# Autodesk Inventor assembly: Wine Rack and Light Shelf Assembly
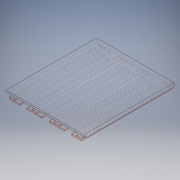
[picture p0: Inventor's stored thumbnail of the model, 180x180]
Saved by Autodesk Inventor 2016 (Build 200138000, 138)
## iProperties
Created: 2017-11-04
Part Number: Wine Rack and Light Shelf Assembly
Document SubType Name: Assembly
Designer: mathaetaes
Author: mathaetaes
## Documents named in this file (4)
- E:\Projects\3D Printer\printer projects\My Designs\Bar Cabinet 2.2.2018\Wine Rack and Light Shelf Assembly Left.iam
- E:\Projects\3D Printer\printer projects\My Designs\Bar Cabinet 2.2.2018\Wine Glass Rack Edge.iam
- E:\Projects\3D Printer\printer projects\My Designs\Bar Cabinet 2.2.2018\Wine Glass Rack Middle.iam
- E:\Projects\3D Printer\printer projects\My Designs\Bar Cabinet 2.2.2018\Horizontal Shelf with Lights Left.ipt
## Components (5 placed, 3 different names)
1. Wine Glass Rack Edge:1 [sub-assembly] — Flush:5, Flush:12, Mate:1
2. Wine Glass Rack Middle:1 [sub-assembly] — Flush:6, Flush:11, Mate:2
3. Wine Glass Rack Edge:2 [sub-assembly] — Flush:8, Flush:9, Mate:4
4. Wine Glass Rack Middle:2 [sub-assembly] — Flush:7, Flush:10, Mate:3
5. Horizontal Shelf with Lights Left:1 — Flush:5, Flush:6, Flush:7, Flush:8, Flush:9, Flush:10, Flush:11, Flush:12, Mate:1, Mate:2, Mate:3, Mate:4
## Relationships (12: Flush 8, Mate 4)
- Flush:5: Wine Glass Rack Edge:1 ↔ Horizontal Shelf with Lights Left:1
- Flush:6: Wine Glass Rack Middle:1 ↔ Horizontal Shelf with Lights Left:1
- Flush:7: Wine Glass Rack Middle:2 ↔ Horizontal Shelf with Lights Left:1
- Flush:8: Wine Glass Rack Edge:2 ↔ Horizontal Shelf with Lights Left:1
- Flush:9: Wine Glass Rack Edge:2 ↔ Horizontal Shelf with Lights Left:1
- Flush:10: Wine Glass Rack Middle:2 ↔ Horizontal Shelf with Lights Left:1
- Flush:11: Wine Glass Rack Middle:1 ↔ Horizontal Shelf with Lights Left:1
- Flush:12: Wine Glass Rack Edge:1 ↔ Horizontal Shelf with Lights Left:1
- Mate:1: Wine Glass Rack Edge:1 ↔ Horizontal Shelf with Lights Left:1
- Mate:2: Wine Glass Rack Middle:1 ↔ Horizontal Shelf with Lights Left:1
- Mate:3: Wine Glass Rack Middle:2 ↔ Horizontal Shelf with Lights Left:1
- Mate:4: Wine Glass Rack Edge:2 ↔ Horizontal Shelf with Lights Left:1
